# Autodesk Inventor assembly: Whole thing
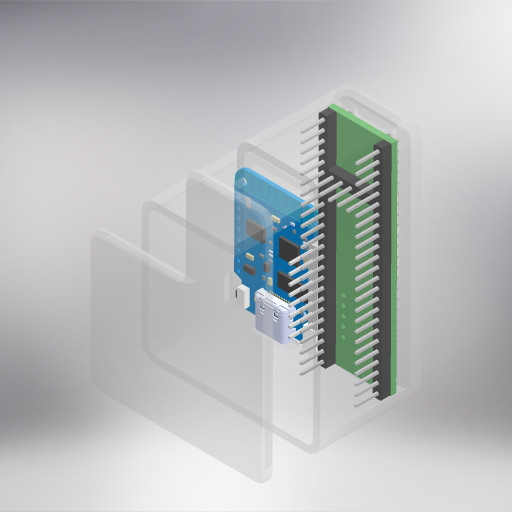
[picture p0: Inventor's stored thumbnail of the model, 512x512]
Saved by Autodesk Inventor 2024 (Build 280153000, 153)
## iProperties
Created: 2024-10-30
Part Number: Whole thing
Document SubType Name: Assembly
Designer: Tejas
Author: Tejas
## Documents named in this file (5)
- C:\Users\Tejas\Documents\Uni 2024 T3\COMP6841\CAD\Whole thing.iam
- C:\Users\Tejas\Documents\Uni 2024 T3\COMP6841\CAD\Teensy 3.5 - 3.6\Teensy 3.5 - 3.6.iam
- C:\Users\Tejas\Documents\Uni 2024 T3\COMP6841\CAD\wemos d1 mini V4\wemos d1 mini V4.iam
- C:\Users\Tejas\Documents\Uni 2024 T3\COMP6841\CAD\Case.ipt
- C:\Users\Tejas\Documents\Uni 2024 T3\COMP6841\CAD\Case Top.ipt
## Components (4 placed, 4 different names)
1. Teensy 3.5 - 3.6:1 [sub-assembly] — Mate:1, Flush:1
2. wemos d1 mini V4:1 [sub-assembly] — Mate:1
3. Case:1 — Flush:1
4. Case Top:1
## Relationships (2: Mate 1, Flush 1)
- Mate:1: Teensy 3.5 - 3.6:1 ↔ wemos d1 mini V4:1
- Flush:1: Teensy 3.5 - 3.6:1 ↔ Case:1
